# Autodesk Inventor assembly: BL Motor + Encoder + Gearbox
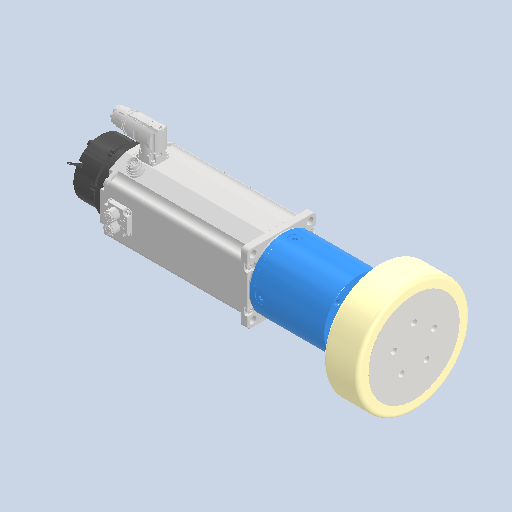
[picture p0: Inventor's stored thumbnail of the model, 512x512]
Saved by Autodesk Inventor 2022.1 (Build 261234000, 234)
## iProperties
Created: 2021-09-22
Part Number: BL Motor + Encoder + Gearbox
Document SubType Name: Assembly
Designer: seb_0
Author: seb_0
## Documents named in this file (6)
- C:\Users\seb_0\Desktop\PDM\BL Motor + Encoder + Gearbox + Rueda.iam
- C:\Users\seb_0\Desktop\PDM\BL Motor - BG 95X80 dPro PN\bg-95x80-885950680018.iam
- C:\Users\seb_0\Desktop\PDM\Encoder - E 600R\e600-8871002100.ipt
- C:\Users\seb_0\Desktop\PDM\Gearbox - PLG 90 HT 10.1\plg-95-8889505003.ipt
- C:\Users\seb_0\Desktop\PDM\Rueda\Rueda.iam
- C:\Users\seb_0\Desktop\PDM\Rueda\Sprocket_Rueda.ipt
## Components (5 placed, 5 different names)
1. bg-95x80-885950680018:1 [sub-assembly] — Coincidencia:1, Coincidencia:2, Coincidencia:3, Coincidencia:4, Coincidencia:5, Coincidencia:6, Coincidencia:7, Coincidencia:8
2. e600-8871002100:1 — Coincidencia:3, Coincidencia:4, Coincidencia:5
3. plg-95-8889505003:1 — Coincidencia:6, Coincidencia:7, Coincidencia:8, Coincidencia:9, Coincidencia:10, Nivelación:1
4. Rueda:1 [sub-assembly] — Coincidencia:11, Coincidencia:12, Coincidencia:13
5. Sprocket_Rueda:1 — Coincidencia:9, Coincidencia:10, Nivelación:1, Coincidencia:11, Coincidencia:12, Coincidencia:13
## Relationships (14: Mate 13, Flush 1)
- Coincidencia:1 [Mate]: bg-95x80-885950680018:1
- Coincidencia:2 [Mate] (5 mm): bg-95x80-885950680018:1
- Coincidencia:3 [Mate]: bg-95x80-885950680018:1 ↔ e600-8871002100:1
- Coincidencia:4 [Mate]: bg-95x80-885950680018:1 ↔ e600-8871002100:1
- Coincidencia:5 [Mate]: bg-95x80-885950680018:1 ↔ e600-8871002100:1
- Coincidencia:6 [Mate]: bg-95x80-885950680018:1 ↔ plg-95-8889505003:1
- Coincidencia:7 [Mate]: bg-95x80-885950680018:1 ↔ plg-95-8889505003:1
- Coincidencia:8 [Mate] (27.5 mm): bg-95x80-885950680018:1 ↔ plg-95-8889505003:1
- Coincidencia:9 [Mate]: plg-95-8889505003:1 ↔ Sprocket_Rueda:1
- Coincidencia:10 [Mate]: plg-95-8889505003:1 ↔ Sprocket_Rueda:1
- Nivelación:1 [Flush]: plg-95-8889505003:1 ↔ Sprocket_Rueda:1
- Coincidencia:11 [Mate]: Rueda:1 ↔ Sprocket_Rueda:1
- Coincidencia:12 [Mate]: Rueda:1 ↔ Sprocket_Rueda:1
- Coincidencia:13 [Mate]: Rueda:1 ↔ Sprocket_Rueda:1
